# Autodesk Inventor assembly: 0072-DXP(F,D-26690)
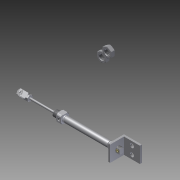
[picture p0: Inventor's stored thumbnail of the model, 180x180]
Saved by Autodesk Inventor 2012 (Build 160160000, 160)
## iProperties
Category: PARTsolutions
Company: BIMBA
Created: 2013-01-17
Part Number: 0072-DXP(F,D-26690)
Catalog Web Link: www.cadenas.de
Description: Original Line Standard Air Cylinders-
Vendor: BIMBA
Document SubType Name: Assembly
Designer: William
Manufacturer: BIMBA
PSOL_IDENT_0: {\\10.0.0.242\data_v9\23d-libs\bimba\bimba\bimba_imperial\bimba_full_line\original_line_cylinders\st
PSOL_IDENT_1: andard_air_cylinders\standard_air_cylinder_asmtab.prj},318 {VTYP=3D},{STYP=ASSTAB},{NB=0072-DXP(F,D-
PSOL_IDENT_2: 26690)},{LINA=0072-DXP},{NN=Original Line Standard Air Cylinders},{DATE=06.09.2012 11:26:56},{GEOMDA
PSOL_IDENT_3: TE=06.09.2012},{VERSION=},{LINEID=20},{LINESUBID=-1},{WBVAR=STROKE,ACTING,MNT,DER,NR,BM,CO,OO,VO,M,E
PSOL_IDENT_4: E,EEL,K,Q,Y,G,T,B,H,SER,SR,NT,W,HL,STPT1,STPT2,STPT3,STPT4,MB,PB,PRC,TB,MN}  {NB=0072-DXP(F,D-26690)
PSOL_IDENT_5: },{LINA=0072-DXP},{KT=DUMMY},{PN=0072-DXP},{PNC=0072-DXP(F,D-26690)},{PNA=(D-26690)},{DASH=-},{BORE1
PSOL_IDENT_6: =0.31250000},{BORE=5/16\" (007)},{BOREPN=007},{STROKE=2.000},{STROKEALG=[0.011:50/0.001]},{STROKE1=2
PSOL_IDENT_7: .000},{ACTING=D},{ACTINGALG= '' , 'Single Acting (SA)' , 'R' , 'Reverse Single Acting (SA)' , 'D' ,
PSOL_IDENT_8: 'Double Acting (SA)' },{ACTINGPN=D},{MNT=XP},{MNTALG= '' , 'Front Nose Mounting (SA)' , 'XP' , 'Doub
PSOL_IDENT_9: le End or Rear Pivot Mounting (SA)' , 'BF' , 'Front Block Mounting (SA)' },{TYPE=},{MNTPN=XP},{DER=}
PSOL_IDENT_10: ,{DERALG= '' , 'N/A' },{NR=},{NRALG= '' , 'N/A' },{NRPN=},{BM=},{BMALG= '' , 'N/A' },{BMPN=},{CO=},{
PSOL_IDENT_11: COALG= '' , 'N/A' },{OO=},{OOALG= '', 'N/A' },{OOPN=},{VO=Z},{VOALG= 'Z' , 'N/A' },{VOPN=},{OOVOPN=}
PSOL_IDENT_12: ,{M=},{MALG= '', 'Without Magnet', 'M', 'With Magnet' },{EE=},{EEL=0.000},{EEMAX=48.0000},{EEALG= ''
PSOL_IDENT_13: , 'Without Extra Extension', 'EE', 'With Extra Extension' },{EELALG=0},{EEPN=},{EEPN1=0.000},{K=},{K
PSOL_IDENT_14: ALG= '', 'Standard' , 'K' , 'Ports Rotated 90deg K' },{KPN=},{Q=},{QALG= '' , 'N/A' },{QPN=},{Y=},{Y
PSOL_IDENT_15: ALG= '' , 'With Pivot Bushing' },{YPN=},{YCON=Y},{F=},{FALG= '', 'Non-Coated (Standard)', 'F', 'Moly
PSOL_IDENT_16: coated' },{FPN=},{G=},{GPN=},{GPN99=},{T=},{TALG= '' , 'Standard -20° to 200°F (-29° to 95°C)' , 'N'
PSOL_IDENT_17: , 'Low Temperature' , 'V' , 'High Temperature' },{NPN=},{VPN=},{B=},{BALG= '' , 'Standard Bumpers'
PSOL_IDENT_18: },{BPN=},{H=},{HALG= '', 'N/A' },{HPN=},{SER=},{SERALG= '' , 'Without Spring Extend/Return' , 'JS' ,
PSOL_IDENT_19: 'With Spring Return' , 'JR' , 'With Spring Extend' },{SR=},{SRALG= '' , 'Standard Stainless Steel'
PSOL_IDENT_20: },{SRPN=},{SRCON=0},{NT=},{NTPN=},{W=},{WALG= '' , 'Without Wiper' , 'W' , 'With Wiper' },{WPN=},{E=
PSOL_IDENT_21: },{EALG= '' , 'Standard Seals/Lube' , 'E' , 'Non-Lube Seals/Lube' },{EPN=},{HL=},{HLALG= '' , 'Witho
PSOL_IDENT_22: ut Low Pressure Hydraulic' , 'HL' , 'With Low Pressure Hydraulic' },{ST=},{STALG= '' , 'N/A' },{STPT
PSOL_IDENT_23: 1=},{STPT1ALG= '' , 'N/A' },{STPT2=},{STPT2ALG= '' , 'N/A' },{STPT3=},{STPT3ALG= '' , 'N/A' },{STPT4
PSOL_IDENT_24: =},{STPT4ALG= '' , 'N/A' },{STPN=},{MB=},{MBALG= '' , 'Without Mounting Bracket' , 'F,D-26765' , 'D-
PSOL_IDENT_25: 26765 (front)'  , 'R,D-26765' , 'D-26765 (rear)' , '2x,D-26765' , 'D-26765 (front & rear)'},{MBPN=},
PSOL_IDENT_26: {MBPNALL=D-26765},{MBPNALLREAR=D-26765},{PB=},{PBALG= '' , 'Without Pivot Bracket' , 'D-26689' , 'D-
PSOL_IDENT_27: 26689' },{PBPN=},{PBPNALL=D-26689},{PRC=F,D-26690},{PRCALG= '' , 'W/out Pivot Rod Clevis' , 'F,D-266
PSOL_IDENT_28: 90' , 'D-26690 (front)' },{PRCPN=(F,D-26690)},{PRCPNALL=D-26690},{TB=},{TBALG= '' , 'N/A' },{TBPN=},
PSOL_IDENT_29: {TBPNALL=},{MN=},{MNALG= '' , 'N/A' },{MNPN=},{MNCONF=},{MNCONR=},{TLEN=2.7390},{FRAC=10.0300},{RGCO
PSOL_IDENT_30: N=},{RGDACCON=R},{RHCON=P},{RHCON1=P},{RHCONON=1},{RHACCON=R},{FNUTCON=1},{RNUTCON=1},{FNUTPN=D-801}
PSOL_IDENT_31: ,{RNUTPN=D-801},{FNUTTRANS=0.0000},{RNUTTRANS=0.0000},{VHOLECON=0},{A1=0.8450},{A1N=0.6250},{A1P=0.8
PSOL_IDENT_32: 450},{A1B=0.9060},{A4=0.1585},{A4N=0.2550},{A4P=0.1585},{A5=0.0220},{A1H=0.875},{A1NH=0.3280},{A1PH=
PSOL_IDENT_33: 0.8750},{A1BH=0.0000},{A1SH=0.0000},{A2H=0.1585},{A2NH=0.1585},{LENGTH=2.0300},{LENGTH1=2.0300},{LEN
PSOL_IDENT_34: GTH2=2.0400},{MUL=2.0000},{MUL11=2.0000},{MUL22=5},{MUL33=3.0000},{MUL2=2.0000},{MUL211=2.0000},{MUL
PSOL_IDENT_35: 222=1.2500},{MUL233=0.7500},{SSS=4.0000},{RGLEN=0.7085},{RHLEN=0.5825},{SSS1=4.0000},{A13=0.7190},{D
PSOL_IDENT_36: IF=0.0000},{G5=0.0000},{ON=0},{SSADD=0.0000},{BADD=0.0000},{MADD=0.0000},{NVADD=0.0000},{TRACKL=2.43
PSOL_IDENT_37: 30},{TRACKCON=D-74168},{TRIMCON=0},{TRIMCON1=0},{PINCON=},{FSPACE=0.3896},{SPACE=0.0268},{TEXT=0.046
PSOL_IDENT_38: 9},{S1=0.5000},{D1=0.0000},{D1N=0.3590},{D1B=0.6050},{D1P=0.0000},{FA=0.560},{RA=0.5600},{PPATH=stan
PSOL_IDENT_39: dard_air_cylinder_asmtpl.prj},{MATALGHTML=<b>Standard Original Line:</b><dl><dt>Rod:</dt><dd>- Stain
PSOL_IDENT_40: less Steel</dd><dd>&nbsp;&nbsp;(5/16  9/16 Bores)</dd><dd>- High Strength Carbon Steel</dd><dd>&nbs
PSOL_IDENT_41: p;&nbsp;(3/4  3 Bore)</dd><dd>- Stainless Steel</dd><dd>&nbsp;&nbsp;(X style DXP/DX/DXDE)</dd><d
PSOL_IDENT_42: t>Bearings:</dt><dd>- Sintered Bronze</dd><dt>Body:</dt><dd>- 304 Stainless Steel</dd><dt>End Caps:<
PSOL_IDENT_43: /dt><dd>- Aluminum</dd><dt>Seals:</dt><dd>- Buna N</dd></dl>},{ASSCFGPRA=007DXP},{MBPNA=},{MNPNA=},{
PSOL_IDENT_44: PRCPNA=(D-26690)},{ASSOPTACC=STPT4},{A=4.03},{HADD=0.0000},{WFL=0},{QADD=0.000},{QADD1=0.200},{TEST=
PSOL_IDENT_45: 2.0000},{MNTB=},{STDNUTF=1},{STDNUTR=1}
CNS_NT: Standard Male Thread
CNS_NB: 0072-DXP(F,D-26690)
CNS_NBSYN: $PNC.
CNS_LINA: 0072-DXP
CNS_PN: 0072-DXP
CNS_PNC: 0072-DXP(F,D-26690)
CNS_PNA: (D-26690)
CNS_DASH: -
CNS_BORE1: 0.31250000
CNS_BORE: 5/16" [007]
CNS_BOREPN: 007
CNS_STROKE: 2.000
CNS_STROKEALG: [0.011:50/0.001]
CNS_STROKE1: 2.000
CNS_ACTING: Double [D]
CNS_ACTINGALG: '' , 'Single Acting (SA)' , 'R' , 'Reverse Single Acting (SA)' , 'D' , 'Double Acting (SA)'
CNS_ACTINGPN: D
CNS_MNT: Universal Double End or Rear Pivot [XP]
CNS_MNTALG: '' , 'Front Nose Mounting (SA)' , 'XP' , 'Double End or Rear Pivot Mounting (SA)' , 'BF' , 'Front Block Mounting (SA)'
CNS_MNTPN: XP
CNS_DER: N/A
CNS_DERALG: '' , 'N/A'
CNS_NR: N/A
CNS_NRALG: '' , 'N/A'
CNS_BM: N/A
CNS_BMALG: '' , 'N/A'
CNS_CO: N/A
CNS_COALG: '' , 'N/A'
CNS_OO: N/A
CNS_OOALG: '', 'N/A'
CNS_VO: N/A
CNS_VOALG: 'Z' , 'N/A'
CNS_M: Without Magnet Piston
CNS_MALG: '', 'Without Magnet', 'M', 'With Magnet'
CNS_EE: Standard Rod Extension
CNS_EEL: 0.000
CNS_EEMAX: 48.0000
CNS_EEALG: '', 'Without Extra Extension', 'EE', 'With Extra Extension'
CNS_EELALG: 0
CNS_EEPN1: 0.000
CNS_K: Standard
CNS_KALG: '', 'Standard' , 'K' , 'Ports Rotated 90deg K'
CNS_Q: N/A
CNS_QALG: '' , 'N/A'
CNS_Y: Pivot Bushing [Y]
CNS_YALG: '' , 'With Pivot Bushing'
CNS_YCON: Y
CNS_FALG: '', 'Non-Coated (Standard)', 'F', 'Molycoated'
CNS_G: Standard Grease Lube
CNS_T: Standard -20° to 200°F (-29° to 95°C)
CNS_TALG: '' , 'Standard -20° to 200°F (-29° to 95°C)' , 'N' , 'Low Temperature' , 'V' , 'High Temperature'
CNS_B: Standard Bumpers
CNS_BALG: '' , 'Standard Bumpers'
CNS_H: N/A
CNS_HALG: '', 'N/A'
CNS_SER: Without Failsafe Spring Extend/Return
CNS_SERALG: '' , 'Without Spring Extend/Return' , 'JS' , 'With Spring Return' , 'JR' , 'With Spring Extend'
CNS_SR: Standard Stainless Steel
CNS_SRALG: '' , 'Standard Stainless Steel'
CNS_SRCON: 0
CNS_W: Without Wiper
CNS_WALG: '' , 'Without Wiper' , 'W' , 'With Wiper'
CNS_EALG: '' , 'Standard Seals/Lube' , 'E' , 'Non-Lube Seals/Lube'
CNS_HL: Standard 250 PSI Air
CNS_HLALG: '' , 'Without Low Pressure Hydraulic' , 'HL' , 'With Low Pressure Hydraulic'
CNS_STALG: '' , 'N/A'
CNS_STPT1: N/A
CNS_STPT1ALG: '' , 'N/A'
CNS_STPT2: N/A
CNS_STPT2ALG: '' , 'N/A'
CNS_STPT3: N/A
CNS_STPT3ALG: '' , 'N/A'
CNS_STPT4: N/A
CNS_STPT4ALG: '' , 'N/A'
CNS_MB: Without Mounting Bracket
CNS_MBALG: '' , 'Without Mounting Bracket' , 'F,D-26765' , 'D-26765 (front)'  , 'R,D-26765' , 'D-26765 (rear)' , '2x,D-26765' , 'D-26765 (front & rear)'
CNS_MBPNALL: D-26765
CNS_MBPNALLREAR: D-26765
CNS_PB: Without Pivot Bracket
CNS_PBALG: '' , 'Without Pivot Bracket' , 'D-26689' , 'D-26689'
CNS_PBPNALL: D-26689
CNS_PRC: D-26690 (front)
CNS_PRCALG: '' , 'W/out Pivot Rod Clevis' , 'F,D-26690' , 'D-26690 (front)'
CNS_PRCPN: (F,D-26690)
CNS_PRCPNALL: D-26690
CNS_TB: N/A
CNS_TBALG: '' , 'N/A'
CNS_MN: N/A
CNS_MNALG: '' , 'N/A'
CNS_TLEN: 2.7390
CNS_FRAC: 10.0300
CNS_RGDACCON: R
CNS_RHCON: P
CNS_RHCON1: P
CNS_RHCONON: 1
CNS_RHACCON: R
CNS_FNUTCON: 1
CNS_RNUTCON: 1
CNS_FNUTPN: D-801
CNS_RNUTPN: D-801
CNS_FNUTTRANS: 0.0000
CNS_RNUTTRANS: 0.0000
CNS_VHOLECON: 0
CNS_A1: 0.8450
CNS_A1N: 0.6250
CNS_A1P: 0.8450
CNS_A1B: 0.9060
CNS_A4: 0.1585
CNS_A4N: 0.2550
CNS_A4P: 0.1585
CNS_A5: 0.0220
CNS_A1H: 0.875
CNS_A1NH: 0.3280
CNS_A1PH: 0.8750
CNS_A1BH: 0.0000
CNS_A1SH: 0.0000
CNS_A2H: 0.1585
CNS_A2NH: 0.1585
CNS_LENGTH: 2.0300
CNS_LENGTH1: 2.0300
CNS_LENGTH2: 2.0400
CNS_MUL: 2.0000
CNS_MUL11: 2.0000
CNS_MUL22: 5.000
CNS_MUL33: 3.0000
CNS_MUL2: 2.0000
CNS_MUL211: 2.0000
CNS_MUL222: 1.2500
CNS_MUL233: 0.7500
CNS_SSS: 4.0000
CNS_RGLEN: 0.7085
CNS_RHLEN: 0.5825
CNS_SSS1: 4.0000
CNS_A13: 0.7190
CNS_DIF: 0.0000
CNS_G5: 0.0000
CNS_ON: 0
CNS_SSADD: 0.0000
CNS_BADD: 0.0000
CNS_MADD: 0.0000
CNS_NVADD: 0.0000
CNS_TRACKL: 2.4330
CNS_TRACKCON: D-74168
CNS_TRIMCON: 0
CNS_TRIMCON1: 0
CNS_FSPACE: 0.3896
CNS_SPACE: 0.0268
CNS_TEXT: 0.0469
CNS_S1: 0.5000
CNS_D1: 0.0000
CNS_D1N: 0.3590
CNS_D1B: 0.6050
CNS_D1P: 0.0000
CNS_FA: 0.560
CNS_RA: 0.5600
CNS_PPATH: standard_air_cylinder_asmtpl.prj
CNS_MATALGHTML: <b>Standard Original Line:</b><dl><dt>Rod:</dt><dd>- Stainless Steel</dd><dd>&nbsp;&nbsp;(5/16  9/16 Bores)</dd><dd>- High Strength Carbon Steel</dd><dd>&nbsp;&nbsp;(3/4  3 Bore)</dd><dd>- Stainless Steel</dd><dd>&nbsp;&nbsp;(X style DXP/DX/DXDE)</dd><dt>Bearings:</dt><dd>- Sintered Bronze</dd><dt>Body:</dt><dd>- 304 Stainless Steel</dd><dt>End Caps:</dt><dd>- Aluminum</dd><dt>Seals:</dt><dd>- Buna N</dd></dl>
CNS_ASSCFGPRA: 007DXP
CNS_PRCPNA: (D-26690)
CNS_ASSOPTACC: STPT4
CNS_A: 4.03
CNS_HADD: 0.0000
CNS_WFL: 0.000
CNS_QADD: 0.000
CNS_QADD1: 0.200
CNS_TEST: 2.0000
CNS_STDNUTF: 1
CNS_STDNUTR: 1
SUPPLIER: BIMBA
ARTICLENO: 0072-DXP(F,D-26690)
BOMINFO: 0072-DXP
CREATOR: CADENAS GmbH
Title: 0072-DXP
Author: Cadenas PARTsolutions
## Documents named in this file (13)
- E:\FRC CAD Files\Robot2013\Launcher\Piston\0072-DXP(F,D-26690).iam
- E:\FRC CAD Files\Robot2013\Launcher\Piston\007R000_rod_guide.ipt
- E:\FRC CAD Files\Robot2013\Launcher\Piston\0072-DXP0_rod.ipt
- E:\FRC CAD Files\Robot2013\Launcher\Piston\D-26690-dummy.ipt
- E:\FRC CAD Files\Robot2013\Launcher\Piston\D-26646.ipt
- E:\FRC CAD Files\Robot2013\Launcher\Piston\D-25368.ipt
- E:\FRC CAD Files\Robot2013\Launcher\Piston\D-25369.ipt
- E:\FRC CAD Files\Robot2013\Launcher\Piston\D-3745.ipt
- E:\FRC CAD Files\Robot2013\Launcher\Piston\007R-2_7390.ipt
- E:\FRC CAD Files\Robot2013\Launcher\Piston\007P0Y000_rear_head.ipt
- E:\FRC CAD Files\Robot2013\Launcher\Piston\D-801.ipt
- E:\FRC CAD Files\Robot2013\Launcher\Piston\D-25359.ipt
- C:\Users\William\Desktop\FRC CAD Files\Robot2013\Launcher\Piston Mounting Bracket.ipt
## Components (14 placed, 12 different names)
1. 007R000_rod_guide:1 — rod_guide_Z@1 <-> rod_cp_Z@2, to_tube_XY@1 <-> tube_front_XY@9, to_tube_Z@1 <-> tube_front_Z@9, to_tube_YZ@1 <-> tube_front_YZ@9
2. 0072-DXP0_rod:1 — rod_guide_Z@1 <-> rod_cp_Z@2, Mate:27, Flush:4
3. D-26690-dummy:1
4. 007R-2_7390:1 — to_tube_XY@1 <-> tube_front_XY@9, to_tube_Z@1 <-> tube_front_Z@9, to_tube_YZ@1 <-> tube_front_YZ@9, tube_rear_XY@9 <-> to_tube_XY@10, tube_rear_Z@9 <-> to_tube_Z@10, tube_rear_YZ@9 <-> to_tube_YZ@10
5. 007P0Y000_rear_head:1 — tube_rear_XY@9 <-> to_tube_XY@10, tube_rear_Z@9 <-> to_tube_Z@10, tube_rear_YZ@9 <-> to_tube_YZ@10, to_pin_XY@10 <-> bushing_XY@12, to_pin_Z@10 <-> bushing_Z@12, to_pin_YZ@10 <-> bushing_YZ@12, Flush:5, Mate:28
6. D-25359:1 — to_pin_XY@10 <-> bushing_XY@12, to_pin_Z@10 <-> bushing_Z@12, to_pin_YZ@10 <-> bushing_YZ@12
7. D-26646:1 — Mate:19, Mate:20, Mate:23, Mate:25, Mate:26, Angle:7
8. D-25368:1 — Mate:19, Mate:21, Mate:22, Mate:24
9. D-25369:1 — Mate:20, Mate:21, Mate:22
10. D-25369:2 — Mate:23, Mate:24
11. D-3745:1 — Mate:25, Mate:26, Angle:7, Mate:27, Flush:4
12. D-801:1
13. D-801:2
14. Piston Mounting Bracket:1 — Flush:5, Mate:28
## Relationships (23: Mate 15, Flush 4, Angle 4)
- rod_guide_Z@1 <-> rod_cp_Z@2 [Mate]: 007R000_rod_guide:1 ↔ 0072-DXP0_rod:1
- to_tube_XY@1 <-> tube_front_XY@9 [Flush]: 007R000_rod_guide:1 ↔ 007R-2_7390:1
- to_tube_Z@1 <-> tube_front_Z@9 [Mate]: 007R000_rod_guide:1 ↔ 007R-2_7390:1
- to_tube_YZ@1 <-> tube_front_YZ@9 [Angle] (0 deg): 007R000_rod_guide:1 ↔ 007R-2_7390:1
- tube_rear_XY@9 <-> to_tube_XY@10 [Flush]: 007R-2_7390:1 ↔ 007P0Y000_rear_head:1
- tube_rear_Z@9 <-> to_tube_Z@10 [Mate]: 007R-2_7390:1 ↔ 007P0Y000_rear_head:1
- tube_rear_YZ@9 <-> to_tube_YZ@10 [Angle] (0 deg): 007R-2_7390:1 ↔ 007P0Y000_rear_head:1
- to_pin_XY@10 <-> bushing_XY@12 [Mate]: 007P0Y000_rear_head:1 ↔ D-25359:1
- to_pin_Z@10 <-> bushing_Z@12 [Mate]: 007P0Y000_rear_head:1 ↔ D-25359:1
- to_pin_YZ@10 <-> bushing_YZ@12 [Angle] (0 deg): 007P0Y000_rear_head:1 ↔ D-25359:1
- Mate:19: D-26646:1 ↔ D-25368:1
- Mate:20: D-26646:1 ↔ D-25369:1
- Mate:21: D-25368:1 ↔ D-25369:1
- Mate:22: D-25368:1 ↔ D-25369:1
- Mate:23: D-26646:1 ↔ D-25369:2
- Mate:24: D-25368:1 ↔ D-25369:2
- Mate:25: D-26646:1 ↔ D-3745:1
- Mate:26: D-26646:1 ↔ D-3745:1
- Angle:7 (0 deg): D-26646:1 ↔ D-3745:1
- Mate:27: 0072-DXP0_rod:1 ↔ D-3745:1
- Flush:4: 0072-DXP0_rod:1 ↔ D-3745:1
- Flush:5: 007P0Y000_rear_head:1 ↔ Piston Mounting Bracket:1
- Mate:28: 007P0Y000_rear_head:1 ↔ Piston Mounting Bracket:1
